# Autodesk Inventor assembly: Ankle
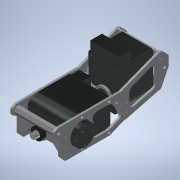
[picture p0: Inventor's stored thumbnail of the model, 180x180]
Saved by Autodesk Inventor 2020 (Build 240168000, 168)
## iProperties
Created: 2016-04-27
Part Number: Ankle
Document SubType Name: Assembly
Designer: hiroaki
Mass: 222.377 g
Surface Area: 394.431 cm^2
Volume: 118.123 cm^3
Density: 1.88259 g/cm^3
Author: hiroaki
## Documents named in this file (13)
- C:\Users\naoki\Documents\Inventor\CitBrains\git_clone\OpenPlatform167\0915\OpenPlatform_ver3_0\LowerBody\Ankle\Ankle.iam
- C:\Users\naoki\Documents\Inventor\CitBrains\git_clone\OpenPlatform167\0915\OpenPlatform_ver3_0\Ready_Made\B3M11xx.ipt
- C:\Users\naoki\Documents\Inventor\CitBrains\git_clone\OpenPlatform167\0915\OpenPlatform_ver3_0\Ready_Made\free_horn.ipt
- C:\Users\naoki\Documents\Inventor\CitBrains\git_clone\OpenPlatform167\0915\OpenPlatform_ver3_0\LowerBody\Ankle\Ankle_side_frame.ipt
- C:\Users\naoki\Documents\Inventor\CitBrains\git_clone\OpenPlatform167\0915\OpenPlatform_ver3_0\LowerBody\Ankle\Ankle_back_frame.ipt
- C:\Users\naoki\Documents\Inventor\CitBrains\git_clone\OpenPlatform167\0915\OpenPlatform_ver3_0\LowerBody\Ankle\Ankle_middle_frame.ipt
- C:\Users\naoki\Documents\Inventor\CitBrains\git_clone\OpenPlatform167\0915\OpenPlatform_ver3_0\LowerBody\Ankle\Ankle_front_frame.ipt
- C:\Users\naoki\Documents\Inventor\CitBrains\git_clone\OpenPlatform167\0915\OpenPlatform_ver3_0\Ready_Made\B3M10xx.ipt
- C:\Users\naoki\Documents\Inventor\CitBrains\git_clone\OpenPlatform167\0915\OpenPlatform_ver3_0\Ready_Made\SLSBF6-39_5-M3-N3.ipt
- C:\Users\naoki\Documents\Inventor\CitBrains\git_clone\OpenPlatform167\0915\OpenPlatform_ver3_0\Ready_Made\BRU-307S.ipt
- C:\Users\naoki\Documents\Inventor\CitBrains\git_clone\OpenPlatform167\0915\OpenPlatform_ver3_0\Ready_Made\S3-07-3W.ipt
- C:\Users\naoki\Documents\Inventor\CitBrains\git_clone\OpenPlatform167\0915\OpenPlatform_ver3_0\Ready_Made\CC-0612-25B.ipt
- C:\Users\naoki\Documents\Inventor\CitBrains\git_clone\OpenPlatform167\0915\OpenPlatform_ver3_0\Ready_Made\UUW-0312-10BH.ipt
## Components (14 placed, 12 different names)
1. B3M11xx:1 — 挿入:23, 挿入:24, 挿入:25, 挿入:26, 挿入:27, 挿入:36, 挿入:51, 挿入:52, 挿入:53
2. B3M10xx:3 — 挿入:42, 挿入:43, 挿入:44, 挿入:45
3. free_horn:1 — 挿入:23
4. Ankle_side_frame:1 — 挿入:24, 挿入:25, 挿入:26, 挿入:27, メイト:1, メイト:2, メイト:3, メイト:4, メイト:5, メイト:6, メイト:8, 挿入:54, 挿入:55
5. Ankle_side_frame:2 — 挿入:36, 挿入:51, 挿入:52, 挿入:53, メイト:9, メイト:10
6. Ankle_back_frame:1 — メイト:1, メイト:2, メイト:3, 挿入:42, 挿入:45
7. Ankle_middle_frame:1 — メイト:4, メイト:5, メイト:6, 挿入:43, 挿入:44
8. Ankle_front_frame:1 — メイト:8, メイト:9, メイト:10, メイト:11, 挿入:58, 挿入:59
9. SLSBF6-39_5-M3-N3:1 — 挿入:54
10. SLSBF6-39_5-M3-N3:2 — 挿入:55
11. BRU-307S:2 — 挿入:60
12. S3-07-3W:1 — メイト:11, 挿入:58
13. CC-0612-25B:1 — 挿入:61
14. UUW-0312-10BH:1 — 挿入:59, 挿入:60, 挿入:61
## Relationships (29: Insert 19, Mate 10)
- 挿入:23 [Insert] (0.2 mm): B3M11xx:1 ↔ free_horn:1
- 挿入:24 [Insert]: B3M11xx:1 ↔ Ankle_side_frame:1
- 挿入:25 [Insert]: B3M11xx:1 ↔ Ankle_side_frame:1
- 挿入:26 [Insert]: B3M11xx:1 ↔ Ankle_side_frame:1
- 挿入:27 [Insert]: B3M11xx:1 ↔ Ankle_side_frame:1
- メイト:1 [Mate] (0.01 mm): Ankle_side_frame:1 ↔ Ankle_back_frame:1
- メイト:2 [Mate]: Ankle_side_frame:1 ↔ Ankle_back_frame:1
- メイト:3 [Mate] (0.01 mm): Ankle_side_frame:1 ↔ Ankle_back_frame:1
- メイト:4 [Mate]: Ankle_side_frame:1 ↔ Ankle_middle_frame:1
- メイト:5 [Mate] (0.01 mm): Ankle_side_frame:1 ↔ Ankle_middle_frame:1
- メイト:6 [Mate] (0.01 mm): Ankle_side_frame:1 ↔ Ankle_middle_frame:1
- 挿入:36 [Insert]: B3M11xx:1 ↔ Ankle_side_frame:2
- メイト:8 [Mate]: Ankle_side_frame:1 ↔ Ankle_front_frame:1
- 挿入:42 [Insert]: B3M10xx:3 ↔ Ankle_back_frame:1
- 挿入:43 [Insert]: B3M10xx:3 ↔ Ankle_middle_frame:1
- 挿入:44 [Insert]: B3M10xx:3 ↔ Ankle_middle_frame:1
- 挿入:45 [Insert]: B3M10xx:3 ↔ Ankle_back_frame:1
- 挿入:51 [Insert]: B3M11xx:1 ↔ Ankle_side_frame:2
- 挿入:52 [Insert]: B3M11xx:1 ↔ Ankle_side_frame:2
- 挿入:53 [Insert]: B3M11xx:1 ↔ Ankle_side_frame:2
- メイト:9 [Mate] (0.01 mm): Ankle_side_frame:2 ↔ Ankle_front_frame:1
- メイト:10 [Mate] (0.01 mm): Ankle_side_frame:2 ↔ Ankle_front_frame:1
- 挿入:54 [Insert]: Ankle_side_frame:1 ↔ SLSBF6-39_5-M3-N3:1
- 挿入:55 [Insert]: Ankle_side_frame:1 ↔ SLSBF6-39_5-M3-N3:2
- メイト:11 [Mate] (0.01 mm): Ankle_front_frame:1 ↔ S3-07-3W:1
- 挿入:58 [Insert]: Ankle_front_frame:1 ↔ S3-07-3W:1
- 挿入:59 [Insert]: Ankle_front_frame:1 ↔ UUW-0312-10BH:1
- 挿入:60 [Insert]: BRU-307S:2 ↔ UUW-0312-10BH:1
- 挿入:61 [Insert]: CC-0612-25B:1 ↔ UUW-0312-10BH:1
